# Autodesk Inventor assembly: extension arm bottom jack
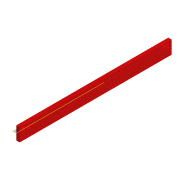
[picture p0: Inventor's stored thumbnail of the model, 180x180]
Saved by Autodesk Inventor 2020 (Build 240168000, 168)
## iProperties
Created: 2019-12-12
Part Number: extension arm bottom jack
Document SubType Name: Assembly
Designer: ball
Author: ball
## Documents named in this file (3)
- C:\FTC\FTC8863CAD\2019 Robot\Delivery\extension arm\extension arm bottom jack.iam
- C:\FTC\FTC8863CAD\2019 Robot\Delivery\extension arm\couple extension arm motor bottom + pulleys.iam
- C:\FTC\FTC8863CAD\2019 Robot\Delivery\extension arm\Coupler extension arm short edited holes for servo.ipt
## Components (2 placed, 2 different names)
1. couple extension arm motor bottom + pulleys:1 [sub-assembly] — Mate:1, Flush:1, Flush:2
2. Coupler extension arm short edited holes for servo:1 — Mate:1, Flush:1, Flush:2
## Relationships (3: Flush 2, Mate 1)
- Mate:1: couple extension arm motor bottom + pulleys:1 ↔ Coupler extension arm short edited holes for servo:1
- Flush:1: couple extension arm motor bottom + pulleys:1 ↔ Coupler extension arm short edited holes for servo:1
- Flush:2: couple extension arm motor bottom + pulleys:1 ↔ Coupler extension arm short edited holes for servo:1
